# Autodesk Inventor assembly: s-assy-gripper_tentioner
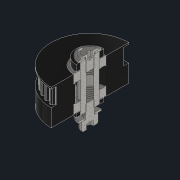
[picture p0: Inventor's stored thumbnail of the model, 180x180]
Saved by Autodesk Inventor 2022 (Build 260153000, 153)
## iProperties
Created: 2021-08-06
Part Number: s-assy-gripper_tentioner
Document SubType Name: Assembly
Designer: yuta0
Mass: 598.977 g
Surface Area: 2161.2 cm^2
Volume: 259.929 cm^3
Density: 2.30439 g/cm^3
Author: yuta0
## Documents named in this file (9)
- C:\Users\yuta0\Documents\GitHub\catchrobo_hardware\assy-robot\s-assy-gripper_tentioner.iam
- C:\Users\yuta0\Documents\GitHub\catchrobo_hardware\assy-robot\base36.ipt
- C:\Users\yuta0\Documents\GitHub\catchrobo_hardware\assy-robot\CB4-6.ipt
- C:\Users\yuta0\Documents\GitHub\catchrobo_hardware\assy-robot\WSJ-STN-M4.ipt
- C:\Users\yuta0\Documents\GitHub\catchrobo_hardware\assy-robot\CBSTSR4-6.ipt
- C:\Users\yuta0\Documents\GitHub\catchrobo_hardware\assy-robot\MR148ZZ.ipt
- C:\Users\yuta0\Documents\GitHub\catchrobo_hardware\assy-robot\ARF-420E.ipt
- C:\Users\yuta0\Documents\GitHub\catchrobo_hardware\assy-robot\base48.ipt
- C:\Users\yuta0\Documents\GitHub\catchrobo_hardware\assy-robot\base47.ipt
## Components (10 placed, 8 different names)
1. WSJ-STN-M4:2 — メイト:87, メイト:127, メイト:128, メイト:144
2. CB4-6:8 — メイト:87, メイト:128, メイト:143, メイト:146
3. CBSTSR4-6:3 — メイト:124, メイト:130, メイト:142
4. WSJ-STN-M4:1 — メイト:124, メイト:130, メイト:145
5. base36:1 — メイト:127, メイト:134, メイト:135, メイト:136, メイト:137, メイト:141
6. MR148ZZ:1 — メイト:134, メイト:135, フラッシュ:1, メイト:147
7. MR148ZZ:2 — メイト:136, メイト:137, メイト:149
8. ARF-420E:1 — メイト:141, メイト:142, メイト:143, メイト:144, フラッシュ:1, メイト:145, メイト:148
9. base48:1 — メイト:146, メイト:147
10. base47:1 — メイト:148, メイト:149
## Relationships (19: Mate 18, Flush 1)
- メイト:87 [Mate]: WSJ-STN-M4:2 ↔ CB4-6:8
- メイト:124 [Mate]: CBSTSR4-6:3 ↔ WSJ-STN-M4:1
- メイト:127 [Mate]: WSJ-STN-M4:2 ↔ base36:1
- メイト:128 [Mate]: WSJ-STN-M4:2 ↔ CB4-6:8
- メイト:130 [Mate]: CBSTSR4-6:3 ↔ WSJ-STN-M4:1
- メイト:134 [Mate]: base36:1 ↔ MR148ZZ:1
- メイト:135 [Mate]: base36:1 ↔ MR148ZZ:1
- メイト:136 [Mate]: base36:1 ↔ MR148ZZ:2
- メイト:137 [Mate]: base36:1 ↔ MR148ZZ:2
- メイト:141 [Mate]: base36:1 ↔ ARF-420E:1
- メイト:142 [Mate]: CBSTSR4-6:3 ↔ ARF-420E:1
- メイト:143 [Mate]: CB4-6:8 ↔ ARF-420E:1
- メイト:144 [Mate] (2 mm): WSJ-STN-M4:2 ↔ ARF-420E:1
- フラッシュ:1 [Flush] (1.6 mm): MR148ZZ:1 ↔ ARF-420E:1
- メイト:145 [Mate]: WSJ-STN-M4:1 ↔ ARF-420E:1
- メイト:146 [Mate]: CB4-6:8 ↔ base48:1
- メイト:147 [Mate]: MR148ZZ:1 ↔ base48:1
- メイト:148 [Mate]: ARF-420E:1 ↔ base47:1
- メイト:149 [Mate]: MR148ZZ:2 ↔ base47:1
